# Autodesk Inventor assembly: MotionBaseGeneric
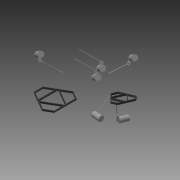
[picture p0: Inventor's stored thumbnail of the model, 180x180]
Saved by Autodesk Inventor 2015 SP1 (Build 190203100, 203)
## iProperties
Created: 2016-02-02
Part Number: MotionBaseGeneric
Document SubType Name: Assembly
Designer: tuttlem
Author: tuttlem
## Documents named in this file (7)
- U:\MotionBase\MotionBaseGeneric.iam
- U:\MotionBase\Platform.ipt
- U:\MotionBase\BasePlatform.ipt
- U:\MotionBase\Rod.ipt
- U:\MotionBase\Rod_MIR.ipt
- U:\MotionBase\arm.ipt
- U:\MotionBase\Motor.ipt
## Components (26 placed, 6 different names)
1. Platform:1 — Insert:3, Insert:5
2. BasePlatform:1
3. Rod:1 — Flush:1, Tangent:1, Insert:3
4. Rod_MIR:1 — Flush:1, Tangent:1, Insert:4
5. Rod:2 — Insert:5
6. Rod_MIR:2 — Insert:6
7. arm:1 — Insert:1, Insert:4
8. Motor:1 — Insert:1
9. arm:8 — Insert:6
10. Motor:7
11. Rod:3
12. Rod_MIR:3
13. arm:9
14. Motor:8
15. Rod:4
16. Rod_MIR:4
17. arm:10
18. Motor:9
19. Rod:5
20. Rod_MIR:5
21. arm:11
22. Motor:10
23. Rod:6
24. Rod_MIR:6
25. arm:12
26. Motor:11
## Relationships (26: Insert 14, Flush 6, Tangent 6)
- Flush:1: Rod:1 ↔ Rod_MIR:1
- Tangent:1: Rod:1 ↔ Rod_MIR:1
- [Flush]: Rod:2 ↔ Rod_MIR:2
- [Tangent]: Rod:2 ↔ Rod_MIR:2
- Insert:1: arm:1 ↔ Motor:1
- [Insert]: arm:8 ↔ Motor:7
- Insert:3: Platform:1 ↔ Rod:1
- Insert:4: Rod_MIR:1 ↔ arm:1
- Insert:5: Platform:1 ↔ Rod:2
- Insert:6: Rod_MIR:2 ↔ arm:8
- [Flush]: Rod:3 ↔ Rod_MIR:3
- [Tangent]: Rod:3 ↔ Rod_MIR:3
- [Insert]: arm:9 ↔ Motor:8
- [Insert]: Rod_MIR:3 ↔ arm:9
- [Flush]: Rod:4 ↔ Rod_MIR:4
- [Tangent]: Rod:4 ↔ Rod_MIR:4
- [Insert]: arm:10 ↔ Motor:9
- [Insert]: Rod_MIR:4 ↔ arm:10
- [Flush]: Rod:5 ↔ Rod_MIR:5
- [Tangent]: Rod:5 ↔ Rod_MIR:5
- [Insert]: arm:11 ↔ Motor:10
- [Insert]: Rod_MIR:5 ↔ arm:11
- [Flush]: Rod:6 ↔ Rod_MIR:6
- [Tangent]: Rod:6 ↔ Rod_MIR:6
- [Insert]: arm:12 ↔ Motor:11
- [Insert]: Rod_MIR:6 ↔ arm:12
## Named parameters: d2_d1 = 0 mm, d3_d0 = 0 mm, d13_d12 = 0 mm, d18_d1 = 0 mm, d19_d12 = 0 mm, d20_d15 = 0 mm, d21_d0 = 0 mm, d22_d1 = 0 mm, d23_d12 = 0 mm, d24_d15 = 0 mm, d25_d0 = 0 mm, d26_d1 = 0 mm, d27_d12 = 0 mm, d28_d15 = 0 mm, d29_d0 = 0 mm, d30_d1 = 0 mm, d31_d12 = 0 mm, d32_d15 = 0 mm, d33_d0 = 0 mm
